# Autodesk Inventor assembly: conmutador redondo M19 conjunto
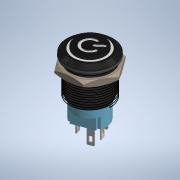
[picture p0: Inventor's stored thumbnail of the model, 180x180]
Saved by Autodesk Inventor 2022 (Build 260153000, 153)
## iProperties
Created: 2021-10-31
Part Number: conmutador redondo M19 conjunto
Document SubType Name: Ensamblaje
Designer: andre
Sending System: SolidWorks 2020
Last Author: ricar
Last Saved: 2021-10-31
Author: andre
## Documents named in this file (7)
- C:\Users\andre\Documents\2021-2\noviembre\ProyectoRobotPallet\base con componentes\boton\conmutador redondo M19 conjunto.iam
- C:\Users\andre\Documents\2021-2\noviembre\ProyectoRobotPallet\base con componentes\boton\conmutador redondo M19 cuerpo.ipt
- C:\Users\andre\Documents\2021-2\noviembre\ProyectoRobotPallet\base con componentes\boton\conmutador redondo M19 aislante trasero.ipt
- C:\Users\andre\Documents\2021-2\noviembre\ProyectoRobotPallet\base con componentes\boton\conmutador redondo M19 pulsador.ipt
- C:\Users\andre\Documents\2021-2\noviembre\ProyectoRobotPallet\base con componentes\boton\conmutador redondo M19 aro interior.ipt
- C:\Users\andre\Documents\2021-2\noviembre\ProyectoRobotPallet\base con componentes\boton\conmutador redondo M19 torica.ipt
- C:\Users\andre\Documents\2021-2\noviembre\ProyectoRobotPallet\base con componentes\boton\tuerca M19x1x2_9.ipt
## Components (6 placed, 6 different names)
1. conmutador redondo M19 cuerpo:1 — Coincidencia:1, Coincidencia:2, Coincidencia:3, Coincidencia:5, Nivelación:1, Coincidencia:7
2. conmutador redondo M19 aislante trasero:1 — Coincidencia:3, Coincidencia:7
3. conmutador redondo M19 pulsador:1 — Coincidencia:4, Coincidencia:6
4. conmutador redondo M19 aro interior:1 — Coincidencia:4, Coincidencia:5, Nivelación:1, Coincidencia:6
5. conmutador redondo M19 torica:1 — Coincidencia:1
6. tuerca M19x1x2_9:1 — Coincidencia:2
## Relationships (8: Mate 7, Flush 1)
- Coincidencia:1 [Mate]: conmutador redondo M19 cuerpo:1 ↔ conmutador redondo M19 torica:1
- Coincidencia:2 [Mate]: conmutador redondo M19 cuerpo:1 ↔ tuerca M19x1x2_9:1
- Coincidencia:3 [Mate]: conmutador redondo M19 cuerpo:1 ↔ conmutador redondo M19 aislante trasero:1
- Coincidencia:4 [Mate]: conmutador redondo M19 pulsador:1 ↔ conmutador redondo M19 aro interior:1
- Coincidencia:5 [Mate]: conmutador redondo M19 cuerpo:1 ↔ conmutador redondo M19 aro interior:1
- Nivelación:1 [Flush]: conmutador redondo M19 cuerpo:1 ↔ conmutador redondo M19 aro interior:1
- Coincidencia:6 [Mate] (-4 mm): conmutador redondo M19 pulsador:1 ↔ conmutador redondo M19 aro interior:1
- Coincidencia:7 [Mate]: conmutador redondo M19 cuerpo:1 ↔ conmutador redondo M19 aislante trasero:1
